# Autodesk Inventor assembly: Jeringa
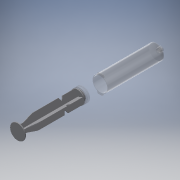
[picture p0: Inventor's stored thumbnail of the model, 180x180]
Saved by Autodesk Inventor 2018.3 (Build 223284000, 284)
## iProperties
Created: 2019-02-26
Part Number: Jeringa
Document SubType Name: Assembly
Designer: Mario
Author: Mario
## Documents named in this file (4)
- C:\Users\Mario\Documents\Inventor\Underwater glider\Jeringa.iam
- C:\Users\Mario\Documents\Inventor\Underwater glider\Jeringa shell.ipt
- C:\Users\Mario\Documents\Inventor\Underwater glider\Jeringa core.ipt
- C:\Users\Mario\Documents\Inventor\Underwater glider\Valvula.ipt
## Components (3 placed, 3 different names)
1. Jeringa shell:1 — Cylindrical:2
2. Jeringa core:1 — Mate:1, Cylindrical:1
3. Valvula:1 — Mate:1, Cylindrical:1, Cylindrical:2
## Relationships (3: CylindricalJoint 2, Mate 1)
- Mate:1: Jeringa core:1 ↔ Valvula:1
- Cylindrical:1: Jeringa core:1 ↔ Valvula:1
- Cylindrical:2: Jeringa shell:1 ↔ Valvula:1
